# Autodesk Inventor assembly: A002
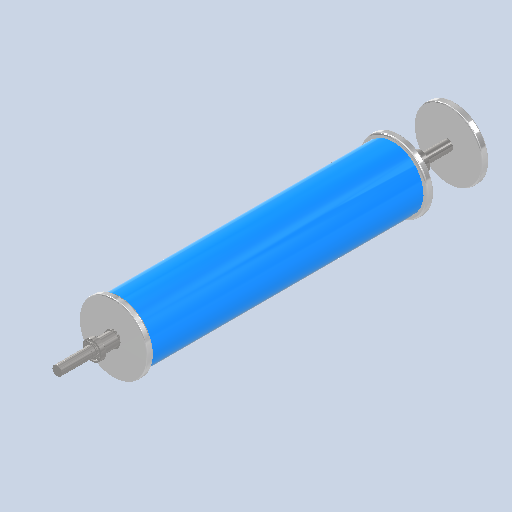
[picture p0: Inventor's stored thumbnail of the model, 512x512]
Saved by Autodesk Inventor 2023 (Build 270158000, 158)
## iProperties
Created: 2022-08-29
Part Number: A002
Document SubType Name: Assembly
Designer: D.C. Eksteen
Author: D.C. Eksteen
Title: POWER ROLLER ASSEMBLY
## Documents named in this file (10)
- C:\Users\dylan\Desktop\Skripsie-2022\Design\CAD\POWER SHAFT ASSEMBLY.iam
- C:\Users\dylan\Desktop\Skripsie-2022\Design\CAD\KEY.ipt
- C:\Users\dylan\Documents\Inventor\Content Center Files\R2023\en-US\STN 022930\STN 022930 - 20.ipt
- C:\Users\dylan\Desktop\Skripsie\WORKSHOP\PARTS\DE STD-0002.ipt
- C:\Users\dylan\Documents\Inventor\Content Center Files\R2023\en-US\STN 022930\STN 022930 - 12.ipt
- C:\Users\dylan\Desktop\Skripsie-2022\Design\CAD\BEARING.ipt
- C:\Users\dylan\Desktop\Skripsie-2022\Design\CAD\POWER ROLLER SHAFT.ipt
- C:\Users\dylan\Desktop\Skripsie-2022\Design\CAD\BRAKE DISC.ipt
- C:\Users\dylan\Desktop\Skripsie-2022\Design\CAD\ROLLER TUBE.ipt
- C:\Users\dylan\Desktop\Skripsie-2022\Design\CAD\POWER ROLLER END CAP.ipt
## Components (15 placed, 9 different names)
1. POWER ROLLER SHAFT:1
2. KEY:1
3. KEY:2 — Mate:18
4. KEY:3 — Mate:20
5. BS 290 SKF- with RS1 seal SKF 61902-RS1:3
6. BS 290 SKF- with RS1 seal SKF 61902-RS1:4
7. BRAKE DISC:1
8. STN 022930 20:1 — Mate:20
9. STN 022930 20:2 — Mate:18
10. STN 022930 15:1
11. STN 022930 15:2
12. STN 022930 12:1
13. ROLLER TUBE:1
14. POWER ROLLER END CAP:1
15. POWER ROLLER END CAP:2
## Relationships (34: Mate 33, Flush 1)
- [Mate]: POWER ROLLER SHAFT:1 ↔ KEY:3
- [Mate]: POWER ROLLER SHAFT:1 ↔ KEY:3
- [Mate]: POWER ROLLER SHAFT:1 ↔ KEY:3
- [Mate]: POWER ROLLER SHAFT:1 ↔ KEY:2
- [Mate]: POWER ROLLER SHAFT:1 ↔ KEY:2
- [Mate]: POWER ROLLER SHAFT:1 ↔ KEY:2
- [Mate]: POWER ROLLER SHAFT:1 ↔ KEY:1
- [Mate]: POWER ROLLER SHAFT:1 ↔ KEY:1
- [Mate]: POWER ROLLER SHAFT:1 ↔ KEY:1
- [Mate]: POWER ROLLER SHAFT:1 ↔ BS 290 SKF- with RS1 seal SKF 61902-RS1:4
- [Mate]: POWER ROLLER SHAFT:1 ↔ BS 290 SKF- with RS1 seal SKF 61902-RS1:4
- [Mate]: POWER ROLLER SHAFT:1 ↔ BS 290 SKF- with RS1 seal SKF 61902-RS1:3
- [Mate]: POWER ROLLER SHAFT:1 ↔ BS 290 SKF- with RS1 seal SKF 61902-RS1:3
- [Mate]: KEY:1 ↔ BRAKE DISC:1
- [Mate]: POWER ROLLER SHAFT:1 ↔ BRAKE DISC:1
- [Mate]: POWER ROLLER SHAFT:1 ↔ BRAKE DISC:1
- [Mate]: POWER ROLLER SHAFT:1 ↔ STN 022930 20:2
- Mate:18: KEY:2 ↔ STN 022930 20:2
- [Mate]: POWER ROLLER SHAFT:1 ↔ STN 022930 20:1
- Mate:20: KEY:3 ↔ STN 022930 20:1
- [Mate]: POWER ROLLER SHAFT:1 ↔ STN 022930 15:1
- [Mate]: POWER ROLLER SHAFT:1 ↔ STN 022930 15:1
- [Mate]: POWER ROLLER SHAFT:1 ↔ STN 022930 15:2
- [Mate]: POWER ROLLER SHAFT:1 ↔ STN 022930 15:2
- [Mate]: POWER ROLLER SHAFT:1 ↔ STN 022930 12:1
- [Mate]: POWER ROLLER SHAFT:1 ↔ STN 022930 12:1
- [Mate]: ROLLER TUBE:1 ↔ POWER ROLLER END CAP:1
- [Mate]: ROLLER TUBE:1 ↔ POWER ROLLER END CAP:1
- [Mate]: ROLLER TUBE:1 ↔ POWER ROLLER END CAP:2
- [Mate]: ROLLER TUBE:1 ↔ POWER ROLLER END CAP:2
- [Mate]: POWER ROLLER SHAFT:1 ↔ POWER ROLLER END CAP:2
- [Mate]: KEY:3 ↔ POWER ROLLER END CAP:1
- [Flush]: KEY:3 ↔ POWER ROLLER END CAP:1
- [Mate]: KEY:2 ↔ POWER ROLLER END CAP:2
